# Autodesk Inventor assembly: Robot
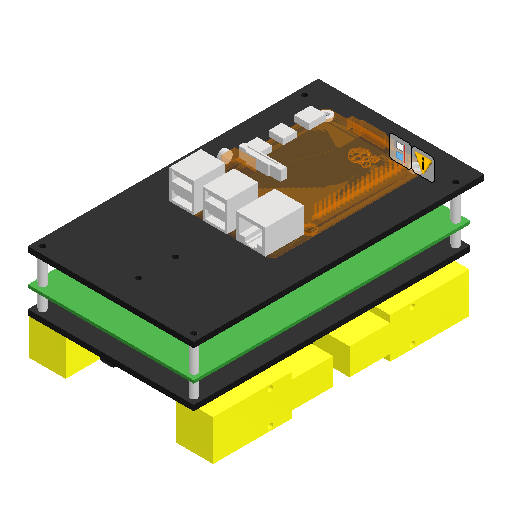
[picture p0: Inventor's stored thumbnail of the model, 512x512]
Saved by Autodesk Inventor 2025.1 (Build 291241000, 241)
## iProperties
Created: 2025-05-09
Part Number: Robot
Document SubType Name: Assembly
Designer: barte
Author: barte
## Documents named in this file (8)
- C:\Users\barte\OneDrive\Dokumenty\Nowy folder\Robot.iam
- C:\Users\barte\OneDrive\Dokumenty\Nowy folder\PCB.ipt
- C:\Users\barte\OneDrive\Dokumenty\Nowy folder\Podstawa.ipt
- C:\Users\barte\OneDrive\Dokumenty\Nowy folder\Podstawa_2.ipt
- C:\Users\barte\OneDrive\Dokumenty\Nowy folder\Silnik.ipt
- C:\Users\barte\OneDrive\Dokumenty\Nowy folder\Dystants.ipt
- C:\Users\barte\OneDrive\Dokumenty\Nowy folder\Dystants2.ipt
- C:\Users\barte\OneDrive\Dokumenty\Nowy folder\Raspberry_Pi_4_B\Raspberry_Pi_4_B\Raspberry_Pi_4_B.ipt
## Components (16 placed, 7 different names)
1. PCB:1 — Zestawiające:24, Zestawiające:25, Zestawiające:26, Zestawiające:27, Zestawiające:28, Zestawiające:30, Zestawiające:32, Zestawiające:33, Zestawiające:34
2. Podstawa:1 — Zestawiające:1, Zestawiające:2, Równoległe:1, Zestawiające:4, Zestawiające:5, Zestawiające:6, Zestawiające:7, Zestawiające:10, Zestawiające:11, Zestawiające:12, Zestawiające:13, Zestawiające:14, Zestawiające:15, Zestawiające:16, Zestawiające:17, Zestawiające:18, Zestawiające:19, Zestawiające:20, Zestawiające:21, Zestawiające:22, Zestawiające:23, Zestawiające:29, Zestawiające:31, Zestawiające:35, Zestawiające:36
3. Podstawa_2:1 — Zestawiające:37, Zestawiające:38, Zestawiające:39, Zestawiające:40, Równoległe:2, Równoległe:3
4. Silnik:1 — Zestawiające:7
5. Silnik:2 — Zestawiające:4, Zestawiające:5, Zestawiające:6
6. Silnik:3 — Zestawiające:10, Zestawiające:11, Zestawiające:12
7. Silnik:4 — Zestawiające:13, Zestawiające:14, Zestawiające:15
8. Dystants:1 — Zestawiające:20, Zestawiające:21, Zestawiające:25
9. Dystants:2 — Zestawiające:16, Zestawiające:17, Zestawiające:26
10. Dystants:3 — Zestawiające:18, Zestawiające:19, Zestawiające:27, Zestawiające:28
11. Dystants:4 — Zestawiające:22, Zestawiające:23, Zestawiające:24
12. Dystants2:1 — Zestawiające:29, Zestawiające:30, Zestawiające:38
13. Dystants2:2 — Zestawiające:34, Zestawiające:36, Zestawiające:39
14. Dystants2:3 — Zestawiające:33, Zestawiające:35, Zestawiające:37
15. Dystants2:4 — Zestawiające:31, Zestawiające:32
16. Raspberry_Pi_4_B:1 — Zestawiające:40, Równoległe:2, Równoległe:3
## Relationships (40: Mate 37, Flush 3)
- Zestawiające:1 [Mate]: Podstawa:1
- Zestawiające:2 [Mate]: Podstawa:1
- Równoległe:1 [Flush]: Podstawa:1
- Zestawiające:4 [Mate]: Podstawa:1 ↔ Silnik:2
- Zestawiające:5 [Mate]: Podstawa:1 ↔ Silnik:2
- Zestawiające:6 [Mate]: Podstawa:1 ↔ Silnik:2
- Zestawiające:7 [Mate]: Podstawa:1 ↔ Silnik:1
- Zestawiające:10 [Mate]: Podstawa:1 ↔ Silnik:3
- Zestawiające:11 [Mate]: Podstawa:1 ↔ Silnik:3
- Zestawiające:12 [Mate]: Podstawa:1 ↔ Silnik:3
- Zestawiające:13 [Mate]: Podstawa:1 ↔ Silnik:4
- Zestawiające:14 [Mate]: Podstawa:1 ↔ Silnik:4
- Zestawiające:15 [Mate]: Podstawa:1 ↔ Silnik:4
- Zestawiające:16 [Mate]: Podstawa:1 ↔ Dystants:2
- Zestawiające:17 [Mate]: Podstawa:1 ↔ Dystants:2
- Zestawiające:18 [Mate]: Podstawa:1 ↔ Dystants:3
- Zestawiające:19 [Mate]: Podstawa:1 ↔ Dystants:3
- Zestawiające:20 [Mate]: Podstawa:1 ↔ Dystants:1
- Zestawiające:21 [Mate]: Podstawa:1 ↔ Dystants:1
- Zestawiające:22 [Mate]: Podstawa:1 ↔ Dystants:4
- Zestawiające:23 [Mate]: Podstawa:1 ↔ Dystants:4
- Zestawiające:24 [Mate]: PCB:1 ↔ Dystants:4
- Zestawiające:25 [Mate]: PCB:1 ↔ Dystants:1
- Zestawiające:26 [Mate]: PCB:1 ↔ Dystants:2
- Zestawiające:27 [Mate]: PCB:1 ↔ Dystants:3
- Zestawiające:28 [Mate]: PCB:1 ↔ Dystants:3
- Zestawiające:29 [Mate]: Podstawa:1 ↔ Dystants2:1
- Zestawiające:30 [Mate]: PCB:1 ↔ Dystants2:1
- Zestawiające:31 [Mate]: Podstawa:1 ↔ Dystants2:4
- Zestawiające:32 [Mate]: PCB:1 ↔ Dystants2:4
- Zestawiające:33 [Mate]: PCB:1 ↔ Dystants2:3
- Zestawiające:34 [Mate]: PCB:1 ↔ Dystants2:2
- Zestawiające:35 [Mate]: Podstawa:1 ↔ Dystants2:3
- Zestawiające:36 [Mate]: Podstawa:1 ↔ Dystants2:2
- Zestawiające:37 [Mate]: Podstawa_2:1 ↔ Dystants2:3
- Zestawiające:38 [Mate]: Podstawa_2:1 ↔ Dystants2:1
- Zestawiające:39 [Mate]: Podstawa_2:1 ↔ Dystants2:2
- Zestawiające:40 [Mate]: Podstawa_2:1 ↔ Raspberry_Pi_4_B:1
- Równoległe:2 [Flush] (-6.5 mm): Podstawa_2:1 ↔ Raspberry_Pi_4_B:1
- Równoległe:3 [Flush] (17 mm): Podstawa_2:1 ↔ Raspberry_Pi_4_B:1
